# Autodesk Inventor assembly: Marco_apm_001-2
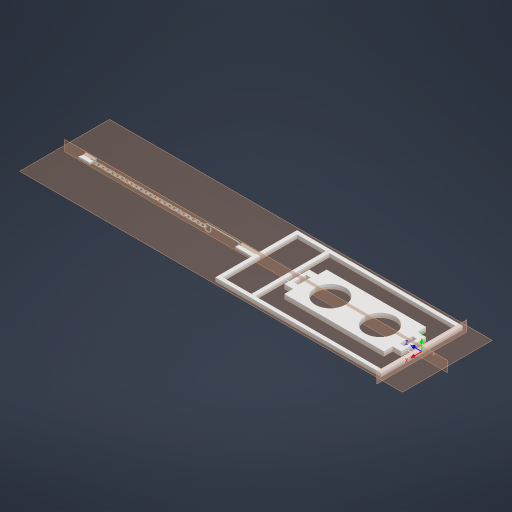
[picture p0: Inventor's stored thumbnail of the model, 512x512]
Saved by Autodesk Inventor 2024 (Build 280153000, 153)
## iProperties
Created: 2023-05-17
Part Number: Marco_apm_001-2
Document SubType Name: Assembly
Designer: javie
Author: javie
## Documents named in this file (5)
- C:\Users\javie\Downloads\Piezas CMR\Marco_APM_001\Marco_apm_001-2.iam
- C:\Users\javie\Downloads\Piezas CMR\Marco_Conveyor_Aereo.iam
- C:\Users\javie\Downloads\Piezas CMR\Marcos_solids\Topes_apm_002-2.ipt
- C:\Users\javie\Downloads\Piezas CMR\Marcos_solids\S_horizontal.ipt
- C:\Users\javie\Downloads\Piezas CMR\Marco_APM_001\Partes\APM_001-2.ipt
## Components (5 placed, 4 different names)
1. Marco_Conveyor_Aereo:1 [sub-assembly] — Insertar:1, Insertar:2
2. Topes_apm_002-2:1 — Insertar:1, Insertar:2, Insertar:3, Insertar:4
3. APM_001-2:1 — Insertar:3, Insertar:4, Insertar:7, Insertar:8
4. S_horizontal:1 — Insertar:5, Insertar:6
5. Topes_apm_002-2:2 — Insertar:5, Insertar:6, Insertar:7, Insertar:8
## Relationships (8: Insert 8)
- Insertar:1: Marco_Conveyor_Aereo:1 ↔ Topes_apm_002-2:1
- Insertar:2: Marco_Conveyor_Aereo:1 ↔ Topes_apm_002-2:1
- Insertar:3: Topes_apm_002-2:1 ↔ APM_001-2:1
- Insertar:4: Topes_apm_002-2:1 ↔ APM_001-2:1
- Insertar:5: S_horizontal:1 ↔ Topes_apm_002-2:2
- Insertar:6: S_horizontal:1 ↔ Topes_apm_002-2:2
- Insertar:7: APM_001-2:1 ↔ Topes_apm_002-2:2
- Insertar:8: APM_001-2:1 ↔ Topes_apm_002-2:2
